# Autodesk Inventor assembly: CL7-200
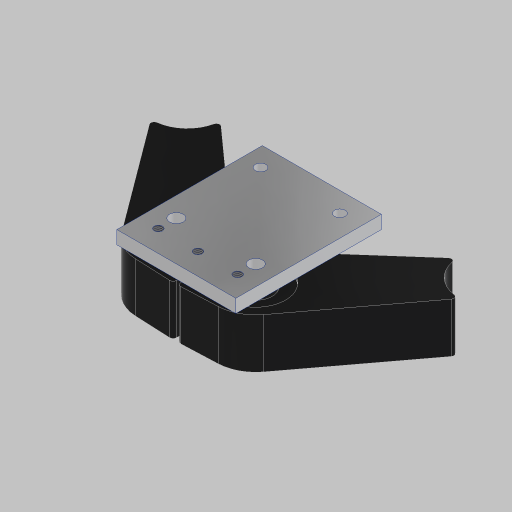
[picture p0: Inventor's stored thumbnail of the model, 512x512]
Saved by Autodesk Inventor 2023.5 (Build 275446000, 446)
## iProperties
Created: 2025-03-17
Part Number: CL7-200
Document SubType Name: Assembly
Designer: dlangdon
Author: dlangdon
## Documents named in this file (4)
- C:\Users\slick\OneDrive\Desktop\2025-ReefScape---CAD\Climber\CL7\CL7-200.iam
- C:\Users\slick\OneDrive\Desktop\2025-ReefScape---CAD\Climber\CL7\CL7-005.ipt
- C:\Users\slick\OneDrive\Desktop\2025-ReefScape---CAD\Climber\CL7\CL7-004.ipt
- C:\Users\slick\OneDrive\Desktop\2025-ReefScape---CAD\Climber\CL7\CL7-005a.ipt
## Components (4 placed, 3 different names)
1. CL7-005:1 — Mate:1, Mate:2, Mate:3, Mate:4, Mate:5, Mate:6
2. CL7-005a:1 — Mate:1, Mate:2, Mate:3
3. CL7-004:1 — Mate:5, Flush:1
4. CL7-004:2 — Mate:4, Mate:6, Flush:1
## Relationships (7: Mate 6, Flush 1)
- Mate:1: CL7-005:1 ↔ CL7-005a:1
- Mate:2: CL7-005:1 ↔ CL7-005a:1
- Mate:3 (25.4 mm): CL7-005:1 ↔ CL7-005a:1
- Mate:4: CL7-005:1 ↔ CL7-004:2
- Mate:5: CL7-005:1 ↔ CL7-004:1
- Mate:6 (1.5875 mm): CL7-005:1 ↔ CL7-004:2
- Flush:1: CL7-004:1 ↔ CL7-004:2
